# Autodesk Inventor assembly: UNLHEP-14-01-A-008_PickerWStamp
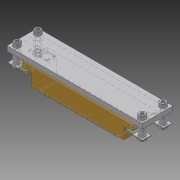
[picture p0: Inventor's stored thumbnail of the model, 180x180]
Saved by Autodesk Inventor 2013 (Build 170138000, 138)
## iProperties
Created: 2014-01-23
Part Number: UNLHEP-14-01-A-008_PickerWStamp
Document SubType Name: Assembly
Designer: Frank Meier
Project: UNL Pixel Phase I
Author: Frank Meier
## Documents named in this file (3)
- C:\Users\Frank Meier\Documents\Inventor\Delvotec-Saugplatte\UNLHEP-14-01-A-008_PickerWStamp.iam
- C:\Users\Frank Meier\Documents\Inventor\Delvotec-Saugplatte\UNLHEP-14-01-A-007_Picker.iam
- C:\Users\Frank Meier\Documents\Inventor\Delvotec-Saugplatte\UNLHEP-14-01-A-006_Rubberstamp.iam
## Components (2 placed, 2 different names)
1. UNLHEP-14-01-A-007_Picker:1 [sub-assembly] — Passend:1
2. UNLHEP-14-01-A-006_Rubberstamp:1 [sub-assembly] — Passend:1
## Relationships (1: Mate 1)
- Passend:1 [Mate]: UNLHEP-14-01-A-007_Picker:1 ↔ UNLHEP-14-01-A-006_Rubberstamp:1
